# Autodesk Inventor assembly: Camera_Autofocus_Mount
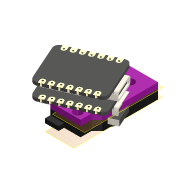
[picture p0: Inventor's stored thumbnail of the model, 180x180]
Saved by Autodesk Inventor 2022 (Build 260153000, 153)
## iProperties
Created: 2023-06-23
Part Number: Camera_Autofocus_Mount
Document SubType Name: Assembly
Designer: diederichbenedict
Author: diederichbenedict
## Documents named in this file (4)
- C:\Users\diederichbenedict\Dropbox\Dokumente\Promotion\PROJECTS\openUC2-CAD\INVENTOR\Camera_Autofocus_Mount.iam
- C:\Users\diederichbenedict\Dropbox\Dokumente\Promotion\PROJECTS\openUC2-CAD\INVENTOR\Jordiscope_XYZ_Case_Printed\30_Linear_Stage_NEMA11_baseholder_bayonetmount_objective_autofocus_kes400_camerabracket_underAnAngle.ipt
- C:\Users\diederichbenedict\Dropbox\Dokumente\Promotion\PROJECTS\openUC2-CAD\INVENTOR\30_Linear_Stage_NEMA11_baseholder_bayonetmount_objective_autofocus_kes400_camerabracket_underAnAngle_counterplate.ipt
- C:\Users\diederichbenedict\Dropbox\Dokumente\Promotion\PROJECTS\openUC2-CAD\INVENTOR\00_Seeeduino Xiao.ipt
## Components (3 placed, 3 different names)
1. 00_Seeeduino Xiao:1 — Winkel:1
2. 30_Linear_Stage_NEMA11_baseholder_bayonetmount_objective_autofocus_kes400_camerabracket_underAnAngle:1 — Fluchtend:1, Fluchtend:2, Winkel:1
3. 30_Linear_Stage_NEMA11_baseholder_bayonetmount_objective_autofocus_kes400_camerabracket_underAnAngle_counterplate:1 — Fluchtend:1, Fluchtend:2
## Relationships (4: Flush 2, Insert 1, Angle 1)
- Fluchtend:1 [Flush]: 30_Linear_Stage_NEMA11_baseholder_bayonetmount_objective_autofocus_kes400_camerabracket_underAnAngle:1 ↔ 30_Linear_Stage_NEMA11_baseholder_bayonetmount_objective_autofocus_kes400_camerabracket_underAnAngle_counterplate:1
- Fluchtend:2 [Flush]: 30_Linear_Stage_NEMA11_baseholder_bayonetmount_objective_autofocus_kes400_camerabracket_underAnAngle:1 ↔ 30_Linear_Stage_NEMA11_baseholder_bayonetmount_objective_autofocus_kes400_camerabracket_underAnAngle_counterplate:1
- [Insert]: 00_Seeeduino Xiao:1 ↔ 30_Linear_Stage_NEMA11_baseholder_bayonetmount_objective_autofocus_kes400_camerabracket_underAnAngle:1
- Winkel:1 [Angle] (180 deg): 00_Seeeduino Xiao:1 ↔ 30_Linear_Stage_NEMA11_baseholder_bayonetmount_objective_autofocus_kes400_camerabracket_underAnAngle:1
